# Autodesk Inventor assembly: rotating_table
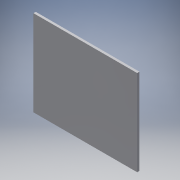
[picture p0: Inventor's stored thumbnail of the model, 180x180]
Saved by Autodesk Inventor 2016 (Build 200138000, 138)
## iProperties
Created: 2016-05-10
Part Number: rotating_table
Document SubType Name: Assembly
Designer: MAS Staff
Author: MAS Staff
## Documents named in this file (4)
- C:\Users\MAS Staff\Desktop\robocup-at-work\models\arena\elements\devices\rotating_turntable\inventor\rotating_table.iam
- C:\Users\MAS Staff\Desktop\robocup-at-work\models\arena\elements\devices\rotating_turntable\inventor\rotating_table_bottom_plate.ipt
- C:\Users\MAS Staff\Desktop\robocup-at-work\models\arena\elements\devices\rotating_turntable\inventor\rotating_table_shaft_plate.ipt
- C:\Users\MAS Staff\Desktop\robocup-at-work\models\arena\elements\devices\rotating_turntable\inventor\rotating_table_shaft.ipt
## Components (3 placed, 3 different names)
1. rotating_table_bottom_plate:1 — Mate:1, Mate:2, Mate:3
2. rotating_table_shaft_plate:1 — Mate:1, Mate:2, Mate:3, Mate:4, Mate:5
3. rotating_table_shaft:1 — Mate:4, Mate:5
## Relationships (5: Mate 5)
- Mate:1: rotating_table_bottom_plate:1 ↔ rotating_table_shaft_plate:1
- Mate:2 (353.55 mm): rotating_table_bottom_plate:1 ↔ rotating_table_shaft_plate:1
- Mate:3 (-353.55 mm): rotating_table_bottom_plate:1 ↔ rotating_table_shaft_plate:1
- Mate:4: rotating_table_shaft_plate:1 ↔ rotating_table_shaft:1
- Mate:5: rotating_table_shaft_plate:1 ↔ rotating_table_shaft:1
